# Autodesk Inventor assembly: E001_BancDeTest
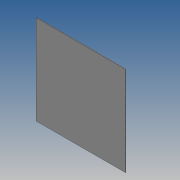
[picture p0: Inventor's stored thumbnail of the model, 180x180]
Saved by Autodesk Inventor 2021.3 (Build 253353000, 353)
## iProperties
Created: 2021-09-24
Part Number: E001_BancDeTest
Document SubType Name: Assembly
Designer: gabri
Author: gabri
## Documents named in this file (4)
- D:\PGA\E001_BancDeTest.iam
- D:\PGA\P002_plancher.ipt
- D:\PGA\P003_tripod.ipt
- D:\PGA\P004_CageDeTest2.ipt
## Components (3 placed, 3 different names)
1. P002_plancher:1 — Placage:1, Placage:2, Placage:3, Placage:5, Mate:6
2. P003_tripod:1 — Placage:5
3. P004_CageDeTest2:1 — Mate:6
## Relationships (5: Mate 5)
- Placage:1 [Mate]: P002_plancher:1
- Placage:2 [Mate]: P002_plancher:1
- Placage:3 [Mate]: P002_plancher:1
- Placage:5 [Mate] (900 mm): P002_plancher:1 ↔ P003_tripod:1
- Mate:6: P002_plancher:1 ↔ P004_CageDeTest2:1
